# Autodesk Inventor assembly: XEndLeft
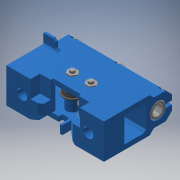
[picture p0: Inventor's stored thumbnail of the model, 180x180]
Saved by Autodesk Inventor 2016 (Build 200138000, 138)
## iProperties
Created: 2014-08-16
Part Number: XEndLeft
Document SubType Name: Assembly
Designer: Jack
Mass: 125.221 g
Surface Area: 373.198 cm^2
Volume: 71.1283 cm^3
Density: 1.76049 g/cm^3
Author: Jack
Title: X End Left
## Documents named in this file (13)
- C:\Users\Jack\ownCloud\Projects\CrossBot\InventorModel\XAxis\XEndLeft.iam
- C:\Users\Jack\ownCloud\Projects\CrossBot\InventorModel\Hardware\Nuts\Nut3.ipt
- C:\Users\Jack\ownCloud\Projects\CrossBot\InventorModel\Hardware\Bolts\SHCS\SHCS4\SHCS4x30.ipt
- C:\Users\Jack\ownCloud\Projects\CrossBot\InventorModel\Hardware\Nuts\Nut4.ipt
- C:\Users\Jack\ownCloud\Projects\CrossBot\InventorModel\Hardware\Bearing\BearingRadialBall\BearingRadialBallF624zz.ipt
- C:\Users\Jack\ownCloud\Projects\CrossBot\InventorModel\Hardware\Wahsers\M4Washer.ipt
- C:\Users\Jack\ownCloud\Projects\CrossBot\InventorModel\Hardware\Bolts\SHCS\SHCS3\SHCS3x8.ipt
- C:\Users\Jack\ownCloud\Projects\CrossBot\InventorModel\XAxis\XAxisBearingSpacer.ipt
- C:\Users\Jack\ownCloud\Projects\CrossBot\InventorModel\Hardware\Bearing\BearingLinear\BearingLinearLMK8.ipt
- C:\Users\Jack\ownCloud\Projects\CrossBot\InventorModel\Hardware\Belt\GT2Idler.iam
- C:\Users\Jack\ownCloud\Projects\CrossBot\InventorModel\XAxis\XAxisBeltIdlerSpacer.ipt
- C:\Users\Jack\ownCloud\Projects\CrossBot\InventorModel\XAxis\XEndLeft.ipt
- C:\Users\Jack\ownCloud\Projects\CrossBot\InventorModel\Hardware\Bolts\SHCS\SHCS3\SHCS3x14.ipt
## Components (26 placed, 12 different names)
1. XAxisBearingSpacer:2 — Mate:51, Mate:52
2. BearingLinearLMK8:1 — Mate:63, Flush:3
3. BearingLinearLMK8:2 — Mate:62, Flush:4
4. GT2Idler:1 [sub-assembly] — Mate:58, Mate:101
5. XAxisBeltIdlerSpacer:1 — Mate:61, Mate:76, Mate:102
6. XEndLeft:1 — Mate:62, Mate:63, Flush:3, Flush:4, Flush:5, Mate:64, Mate:65, Mate:66, Mate:67, Mate:74, Mate:75, Angle:1, Angle:2, Mate:77, Mate:78, Angle:3, Mate:79, Mate:80, Mate:81, Mate:82, Mate:83, Mate:84, Angle:4, Angle:5, Angle:6, Mate:85, Mate:86, Mate:93, Mate:94, Mate:95, Mate:96, Mate:98, Mate:99, Angle:7, Mate:100, Mate:102
7. BearingRadialBallF624zz:3
8. BearingRadialBallF624zz:4
9. M4Washer:4 — Mate:38, Mate:52
10. M4Washer:3 — Mate:79
11. M4Washer:2 — Mate:30, Mate:83
12. M4Washer:1 — Mate:57, Mate:76, Mate:101
13. Nut4:2 — Mate:21, Mate:84, Angle:4
14. Nut4:1 — Mate:20, Mate:78, Angle:3
15. SHCS4x30:2 — Mate:20, Mate:38, Mate:51, Mate:77, Mate:81
16. SHCS4x30:1 — Mate:21, Mate:30, Mate:57, Mate:58, Mate:61, Mate:80, Mate:82
17. Nut3:3 — Mate:43, Angle:5, Mate:86, Flush:7
18. Nut3:4 — Mate:42, Angle:6, Mate:85, Flush:6
19. SHCS3x8:1 — Mate:42, Mate:66, Flush:6
20. SHCS3x8:2 — Mate:43, Mate:67, Flush:7
21. SHCS3x14:2 — Mate:92, Mate:94, Mate:95
22. SHCS3x14:3 — Mate:98, Mate:100
23. Nut3:5 — Mate:99, Angle:7
24. SHCS3x14:1 — Mate:91, Mate:93, Mate:96
25. Nut3:2 — Mate:74, Angle:2, Mate:92
26. Nut3:1 — Mate:75, Angle:1, Mate:91
## Relationships (60: Mate 48, Angle 7, Flush 5)
- Mate:20: Nut4:1 ↔ SHCS4x30:2
- Mate:21: Nut4:2 ↔ SHCS4x30:1
- Mate:30: M4Washer:2 ↔ SHCS4x30:1
- [Mate]: BearingRadialBallF624zz:3 ↔ BearingRadialBallF624zz:4
- [Mate]: BearingRadialBallF624zz:3 ↔ BearingRadialBallF624zz:4
- [Mate]: BearingRadialBallF624zz:3 ↔ M4Washer:3
- [Mate]: BearingRadialBallF624zz:3 ↔ M4Washer:3
- [Mate]: BearingRadialBallF624zz:4 ↔ M4Washer:4
- [Mate]: BearingRadialBallF624zz:4 ↔ M4Washer:4
- Mate:38: M4Washer:4 ↔ SHCS4x30:2
- Mate:42: Nut3:4 ↔ SHCS3x8:1
- Mate:43: Nut3:3 ↔ SHCS3x8:2
- Mate:51: XAxisBearingSpacer:2 ↔ SHCS4x30:2
- Mate:52: XAxisBearingSpacer:2 ↔ M4Washer:4
- Mate:57: M4Washer:1 ↔ SHCS4x30:1
- Mate:58: GT2Idler:1 ↔ SHCS4x30:1
- Mate:61: XAxisBeltIdlerSpacer:1 ↔ SHCS4x30:1
- Mate:62: BearingLinearLMK8:2 ↔ XEndLeft:1
- Mate:63: BearingLinearLMK8:1 ↔ XEndLeft:1
- Flush:3: BearingLinearLMK8:1 ↔ XEndLeft:1
- Flush:4: BearingLinearLMK8:2 ↔ XEndLeft:1
- Flush:5: XEndLeft:1
- Mate:64: XEndLeft:1
- Mate:65: XEndLeft:1
- Mate:66: XEndLeft:1 ↔ SHCS3x8:1
- Mate:67: XEndLeft:1 ↔ SHCS3x8:2
- Mate:74: XEndLeft:1 ↔ Nut3:2
- Mate:75: XEndLeft:1 ↔ Nut3:1
- Angle:1 (0 deg): XEndLeft:1 ↔ Nut3:1
- Angle:2 (0 deg): XEndLeft:1 ↔ Nut3:2
- Mate:76: XAxisBeltIdlerSpacer:1 ↔ M4Washer:1
- Mate:77: XEndLeft:1 ↔ SHCS4x30:2
- Mate:78: XEndLeft:1 ↔ Nut4:1
- Angle:3 (0 deg): XEndLeft:1 ↔ Nut4:1
- Mate:79: XEndLeft:1 ↔ M4Washer:3
- Mate:80: XEndLeft:1 ↔ SHCS4x30:1
- Mate:81: XEndLeft:1 ↔ SHCS4x30:2
- Mate:82: XEndLeft:1 ↔ SHCS4x30:1
- Mate:83: XEndLeft:1 ↔ M4Washer:2
- Mate:84: XEndLeft:1 ↔ Nut4:2
- Angle:4 (0 deg): XEndLeft:1 ↔ Nut4:2
- Angle:5 (0 deg): XEndLeft:1 ↔ Nut3:3
- Angle:6 (0 deg): XEndLeft:1 ↔ Nut3:4
- Mate:85: XEndLeft:1 ↔ Nut3:4
- Mate:86: XEndLeft:1 ↔ Nut3:3
- Flush:6 (-0.5 mm): Nut3:4 ↔ SHCS3x8:1
- Flush:7 (-0.5 mm): Nut3:3 ↔ SHCS3x8:2
- Mate:91: SHCS3x14:1 ↔ Nut3:1
- Mate:92: SHCS3x14:2 ↔ Nut3:2
- Mate:93: XEndLeft:1 ↔ SHCS3x14:1
- Mate:94: XEndLeft:1 ↔ SHCS3x14:2
- Mate:95: XEndLeft:1 ↔ SHCS3x14:2
- Mate:96: XEndLeft:1 ↔ SHCS3x14:1
- [Mate]: SHCS3x14:3 ↔ Nut3:5
- Mate:98: XEndLeft:1 ↔ SHCS3x14:3
- Mate:99: XEndLeft:1 ↔ Nut3:5
- Angle:7 (0 deg): XEndLeft:1 ↔ Nut3:5
- Mate:100: XEndLeft:1 ↔ SHCS3x14:3
- Mate:101: GT2Idler:1 ↔ M4Washer:1
- Mate:102: XAxisBeltIdlerSpacer:1 ↔ XEndLeft:1
## Named parameters: d35_d44 = 0 mm, d36_d45 = 0 mm, d37_d46 = 0 mm, d38_d47 = 0 mm, d39_d48 = 0 mm, d40_d49 = 0 mm, d156_d150 = 0 mm
